# Autodesk Inventor assembly: EnsambleMecanismoEnsayo2
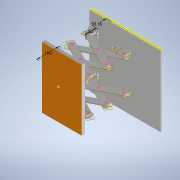
[picture p0: Inventor's stored thumbnail of the model, 180x180]
Saved by Autodesk Inventor 2021 (Build 250183000, 183)
## iProperties
Created: 2021-04-17
Part Number: EnsambleMecanismoEnsayo2
Document SubType Name: Assembly
Designer: GABRIEL LOL
Author: GABRIEL LOL
## Documents named in this file (9)
- J:\PAI\Proyecto_PAI_2021\01 CAD\EnsambleMecanismoEnsayo2.iam
- J:\PAI\Proyecto_PAI_2021\01 CAD\PasadorPivotePreliminar.ipt
- J:\PAI\Proyecto_PAI_2021\01 CAD\PasadorPreliminar.ipt
- J:\PAI\Proyecto_PAI_2021\01 CAD\EslabonPreliminarElevacion.ipt
- J:\PAI\Proyecto_PAI_2021\01 CAD\ApoyoRotatorioPreliminar.ipt
- J:\PAI\Proyecto_PAI_2021\01 CAD\PistaEslabonPreliminar.ipt
- J:\PAI\Proyecto_PAI_2021\01 CAD\SoporteBaseElevacion.ipt
- J:\PAI\Proyecto_PAI_2021\01 CAD\BaseExtrusion.ipt
- J:\PAI\Proyecto_PAI_2021\01 CAD\PisoDeEnsayoIgnorar.ipt
## Components (35 placed, 8 different names)
1. EslabonPreliminarElevacion:1 — Mate:18, Flush:9, Mate:26, Flush:11, Mate:35, Flush:25
2. EslabonPreliminarElevacion:2 — Mate:3, Mate:4, Mate:6, Mate:13, Flush:6, Mate:28, Flush:19
3. EslabonPreliminarElevacion:3 — Mate:12, Flush:5, Mate:25, Flush:10, Mate:30, Flush:21
4. EslabonPreliminarElevacion:4 — Mate:14, Mate:15, Flush:7, Mate:17, Flush:8, Mate:27, Flush:18
5. ApoyoRotatorioPreliminar:3 — Mate:2, Mate:7, Flush:3, Mate:14, Mate:16
6. ApoyoRotatorioPreliminar:4 — Mate:1, Mate:5, Mate:6, Mate:7, Flush:2, Flush:3, Flush:4, Mate:21, Mate:22
7. PasadorPivotePreliminar:3 — Mate:15, Flush:7, Mate:16
8. PasadorPivotePreliminar:4 — Mate:3, Mate:4, Mate:5
9. PasadorPreliminar:2 — Mate:17, Flush:8, Mate:18, Flush:9
10. PasadorPreliminar:3 — Mate:12, Mate:13, Flush:5, Flush:6
11. PistaEslabonPreliminar:1 — Mate:20, Mate:23, Mate:24, Transitional:3, Transitional:4, Flush:37
12. PistaEslabonPreliminar:2 — Mate:19, Mate:21, Mate:22, Mate:23, Mate:24, Transitional:1, Transitional:2, Flush:36
13. SoporteBaseElevacion:1 — Mate:8, Mate:9, Mate:10, Mate:51, Mate:52, Flush:33, Flush:34, Mate:53
14. BaseExtrusion:1 — Mate:8, Mate:9, Mate:10
15. PisoDeEnsayoIgnorar:1 — Mate:1, Mate:2, Flush:2, Flush:4, Mate:19, Mate:20
16. PasadorPreliminar:4 — Mate:25, Flush:10, Transitional:1, Transitional:2
17. PasadorPreliminar:6 — Mate:26, Flush:11, Transitional:3, Transitional:4
18. PasadorPreliminar:7 — Mate:28, Flush:19, Mate:29, Flush:20
19. PasadorPreliminar:8 — Mate:27, Flush:18, Mate:39, Flush:29
20. EslabonPreliminarElevacion:5 — Mate:36, Flush:26, Mate:37, Flush:27, Mate:40, Flush:30
21. EslabonPreliminarElevacion:6 — Mate:29, Flush:20, Mate:34, Mate:41, Mate:44, Mate:46
22. EslabonPreliminarElevacion:7 — Mate:38, Flush:28, Mate:39, Flush:29, Mate:42, Mate:43, Mate:48
23. EslabonPreliminarElevacion:8 — Mate:31, Flush:22, Mate:32, Flush:23, Mate:33, Flush:24
24. PasadorPreliminar:9 — Mate:32, Flush:23, Transitional:7, Transitional:8, Flush:32
25. PasadorPreliminar:10 — Mate:30, Flush:21, Mate:31, Flush:22
26. PasadorPreliminar:11 — Mate:35, Flush:25, Mate:36, Flush:26
27. PasadorPreliminar:12 — Mate:33, Flush:24, Mate:34
28. PasadorPreliminar:14 — Mate:37, Flush:27, Mate:38, Flush:28
29. PasadorPreliminar:15 — Mate:40, Flush:30, Transitional:5, Transitional:6, Flush:31
30. PasadorPivotePreliminar:5 — Mate:42, Mate:43, Mate:47
31. PasadorPivotePreliminar:6 — Mate:41, Mate:44, Mate:45
32. ApoyoRotatorioPreliminar:5 — Mate:45, Mate:46, Mate:53
33. ApoyoRotatorioPreliminar:6 — Mate:47, Mate:48, Mate:52, Flush:33, Flush:34
34. PistaEslabonPreliminar:3 — Transitional:5, Transitional:6, Flush:31, Mate:51, Flush:35, Flush:37
35. PistaEslabonPreliminar:4 — Transitional:7, Transitional:8, Flush:32, Flush:35, Flush:36
## Relationships (88: Mate 50, Flush 30, Transitional 8)
- Mate:1: ApoyoRotatorioPreliminar:4 ↔ PisoDeEnsayoIgnorar:1
- Mate:2: ApoyoRotatorioPreliminar:3 ↔ PisoDeEnsayoIgnorar:1
- Mate:3: EslabonPreliminarElevacion:2 ↔ PasadorPivotePreliminar:4
- Mate:4: EslabonPreliminarElevacion:2 ↔ PasadorPivotePreliminar:4
- Mate:5: ApoyoRotatorioPreliminar:4 ↔ PasadorPivotePreliminar:4
- Mate:6: EslabonPreliminarElevacion:2 ↔ ApoyoRotatorioPreliminar:4
- Mate:7: ApoyoRotatorioPreliminar:3 ↔ ApoyoRotatorioPreliminar:4
- Mate:8: SoporteBaseElevacion:1 ↔ BaseExtrusion:1
- Mate:9: SoporteBaseElevacion:1 ↔ BaseExtrusion:1
- Mate:10: SoporteBaseElevacion:1 ↔ BaseExtrusion:1
- Flush:2: ApoyoRotatorioPreliminar:4 ↔ PisoDeEnsayoIgnorar:1
- Flush:3 (250 mm): ApoyoRotatorioPreliminar:3 ↔ ApoyoRotatorioPreliminar:4
- Flush:4 (108 mm): ApoyoRotatorioPreliminar:4 ↔ PisoDeEnsayoIgnorar:1
- Mate:12: EslabonPreliminarElevacion:3 ↔ PasadorPreliminar:3
- Mate:13: EslabonPreliminarElevacion:2 ↔ PasadorPreliminar:3
- Flush:5: EslabonPreliminarElevacion:3 ↔ PasadorPreliminar:3
- Flush:6: EslabonPreliminarElevacion:2 ↔ PasadorPreliminar:3
- Mate:14: EslabonPreliminarElevacion:4 ↔ ApoyoRotatorioPreliminar:3
- Mate:15: EslabonPreliminarElevacion:4 ↔ PasadorPivotePreliminar:3
- Flush:7: EslabonPreliminarElevacion:4 ↔ PasadorPivotePreliminar:3
- Mate:16: ApoyoRotatorioPreliminar:3 ↔ PasadorPivotePreliminar:3
- Mate:17: EslabonPreliminarElevacion:4 ↔ PasadorPreliminar:2
- Flush:8: EslabonPreliminarElevacion:4 ↔ PasadorPreliminar:2
- Mate:18: EslabonPreliminarElevacion:1 ↔ PasadorPreliminar:2
- Flush:9: EslabonPreliminarElevacion:1 ↔ PasadorPreliminar:2
- Mate:19: PistaEslabonPreliminar:2 ↔ PisoDeEnsayoIgnorar:1
- Mate:20: PistaEslabonPreliminar:1 ↔ PisoDeEnsayoIgnorar:1
- Mate:21: ApoyoRotatorioPreliminar:4 ↔ PistaEslabonPreliminar:2
- Mate:22 (173.4 mm): ApoyoRotatorioPreliminar:4 ↔ PistaEslabonPreliminar:2
- Mate:23: PistaEslabonPreliminar:1 ↔ PistaEslabonPreliminar:2
- Mate:24 (-250 mm): PistaEslabonPreliminar:1 ↔ PistaEslabonPreliminar:2
- Mate:25: EslabonPreliminarElevacion:3 ↔ PasadorPreliminar:4
- Flush:10: EslabonPreliminarElevacion:3 ↔ PasadorPreliminar:4
- Transitional:1: PistaEslabonPreliminar:2 ↔ PasadorPreliminar:4
- Transitional:2: PistaEslabonPreliminar:2 ↔ PasadorPreliminar:4
- Mate:26: EslabonPreliminarElevacion:1 ↔ PasadorPreliminar:6
- Flush:11: EslabonPreliminarElevacion:1 ↔ PasadorPreliminar:6
- Transitional:3: PistaEslabonPreliminar:1 ↔ PasadorPreliminar:6
- Transitional:4: PistaEslabonPreliminar:1 ↔ PasadorPreliminar:6
- Mate:27: EslabonPreliminarElevacion:4 ↔ PasadorPreliminar:8
- Mate:28: EslabonPreliminarElevacion:2 ↔ PasadorPreliminar:7
- Flush:18: EslabonPreliminarElevacion:4 ↔ PasadorPreliminar:8
- Flush:19: EslabonPreliminarElevacion:2 ↔ PasadorPreliminar:7
- Mate:29: PasadorPreliminar:7 ↔ EslabonPreliminarElevacion:6
- Flush:20: PasadorPreliminar:7 ↔ EslabonPreliminarElevacion:6
- Mate:30: EslabonPreliminarElevacion:3 ↔ PasadorPreliminar:10
- Flush:21: EslabonPreliminarElevacion:3 ↔ PasadorPreliminar:10
- Mate:31: EslabonPreliminarElevacion:8 ↔ PasadorPreliminar:10
- Flush:22: EslabonPreliminarElevacion:8 ↔ PasadorPreliminar:10
- Mate:32: EslabonPreliminarElevacion:8 ↔ PasadorPreliminar:9
- Flush:23: EslabonPreliminarElevacion:8 ↔ PasadorPreliminar:9
- Mate:33: EslabonPreliminarElevacion:8 ↔ PasadorPreliminar:12
- Flush:24: EslabonPreliminarElevacion:8 ↔ PasadorPreliminar:12
- Mate:34: EslabonPreliminarElevacion:6 ↔ PasadorPreliminar:12
- Mate:35: EslabonPreliminarElevacion:1 ↔ PasadorPreliminar:11
- Flush:25: EslabonPreliminarElevacion:1 ↔ PasadorPreliminar:11
- Mate:36: EslabonPreliminarElevacion:5 ↔ PasadorPreliminar:11
- Flush:26: EslabonPreliminarElevacion:5 ↔ PasadorPreliminar:11
- Mate:37: EslabonPreliminarElevacion:5 ↔ PasadorPreliminar:14
- Flush:27: EslabonPreliminarElevacion:5 ↔ PasadorPreliminar:14
- Mate:38: EslabonPreliminarElevacion:7 ↔ PasadorPreliminar:14
- Flush:28: EslabonPreliminarElevacion:7 ↔ PasadorPreliminar:14
- Mate:39: PasadorPreliminar:8 ↔ EslabonPreliminarElevacion:7
- Flush:29: PasadorPreliminar:8 ↔ EslabonPreliminarElevacion:7
- Mate:40: EslabonPreliminarElevacion:5 ↔ PasadorPreliminar:15
- Flush:30: EslabonPreliminarElevacion:5 ↔ PasadorPreliminar:15
- Mate:41: EslabonPreliminarElevacion:6 ↔ PasadorPivotePreliminar:6
- Mate:42: EslabonPreliminarElevacion:7 ↔ PasadorPivotePreliminar:5
- Mate:43: EslabonPreliminarElevacion:7 ↔ PasadorPivotePreliminar:5
- Mate:44: EslabonPreliminarElevacion:6 ↔ PasadorPivotePreliminar:6
- Mate:45: PasadorPivotePreliminar:6 ↔ ApoyoRotatorioPreliminar:5
- Mate:46: EslabonPreliminarElevacion:6 ↔ ApoyoRotatorioPreliminar:5
- Mate:47: PasadorPivotePreliminar:5 ↔ ApoyoRotatorioPreliminar:6
- Mate:48: EslabonPreliminarElevacion:7 ↔ ApoyoRotatorioPreliminar:6
- Transitional:5: PasadorPreliminar:15 ↔ PistaEslabonPreliminar:3
- Transitional:6: PasadorPreliminar:15 ↔ PistaEslabonPreliminar:3
- Transitional:7: PasadorPreliminar:9 ↔ PistaEslabonPreliminar:4
- Transitional:8: PasadorPreliminar:9 ↔ PistaEslabonPreliminar:4
- Flush:31: PasadorPreliminar:15 ↔ PistaEslabonPreliminar:3
- Flush:32: PasadorPreliminar:9 ↔ PistaEslabonPreliminar:4
- Mate:51: SoporteBaseElevacion:1 ↔ PistaEslabonPreliminar:3
- Mate:52: SoporteBaseElevacion:1 ↔ ApoyoRotatorioPreliminar:6
- Flush:33: SoporteBaseElevacion:1 ↔ ApoyoRotatorioPreliminar:6
- Flush:34 (105 mm): SoporteBaseElevacion:1 ↔ ApoyoRotatorioPreliminar:6
- Mate:53: SoporteBaseElevacion:1 ↔ ApoyoRotatorioPreliminar:5
- Flush:35: PistaEslabonPreliminar:3 ↔ PistaEslabonPreliminar:4
- Flush:36: PistaEslabonPreliminar:2 ↔ PistaEslabonPreliminar:4
- Flush:37: PistaEslabonPreliminar:1 ↔ PistaEslabonPreliminar:3
